# Autodesk Inventor assembly: Schuppen
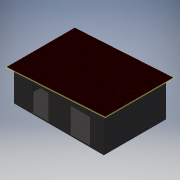
[picture p0: Inventor's stored thumbnail of the model, 180x180]
Saved by Autodesk Inventor 2017 (Build 210142000, 142)
## iProperties
Created: 2017-05-11
Part Number: Schuppen
Document SubType Name: Assembly
Designer: Fake
Author: Fake
## Documents named in this file (4)
- C:\Users\Fake\Documents\Inventor\Oli_Grundstück\Schuppen.iam
- C:\Users\Fake\Documents\Inventor\Oli_Grundstück\Wände.ipt
- C:\Users\Fake\Documents\Inventor\Oli_Grundstück\Grundriss.ipt
- C:\Users\Fake\Documents\Inventor\Oli_Grundstück\Dach.ipt
## Components (3 placed, 3 different names)
1. Grundriss:1 — Fluchtend:1
2. Wände:1 — Fluchtend:1, Fluchtend:2
3. Dach:1 — Fluchtend:2
## Relationships (2: Flush 2)
- Fluchtend:1 [Flush]: Grundriss:1 ↔ Wände:1
- Fluchtend:2 [Flush]: Wände:1 ↔ Dach:1
